# Autodesk Inventor assembly: Montagem1
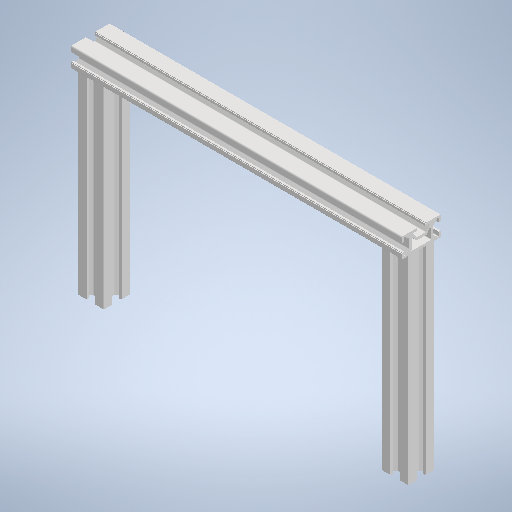
[picture p0: Inventor's stored thumbnail of the model, 512x512]
Saved by Autodesk Inventor 2025.2 (Build 292293000, 293)
## iProperties
Created: 2025-04-08
Part Number: Montagem1
Document SubType Name: Assembly
Designer: kenay
Author: kenay
## Documents named in this file (3)
- C:\Users\kenay\Downloads\Peças\Montagem1.iam
- C:\Users\kenay\Downloads\Peças\Peça3.ipt
- C:\Users\kenay\Downloads\Peças\Peça2.ipt
## Components (3 placed, 2 different names)
1. Peça2:1 — Coincidente:1, Alinhado:4, Coincidente:2, Alinhado:5
2. Peça3:1 — Alinhado:1, Alinhado:2, Alinhado:3, Coincidente:1, Alinhado:4, Alinhado:6, Alinhado:7
3. Peça3:2 — Coincidente:2, Alinhado:5, Alinhado:6, Alinhado:7
## Relationships (9: Flush 7, Mate 2)
- Alinhado:1 [Flush]: Peça3:1
- Alinhado:2 [Flush]: Peça3:1
- Alinhado:3 [Flush]: Peça3:1
- Coincidente:1 [Mate]: Peça2:1 ↔ Peça3:1
- Alinhado:4 [Flush]: Peça2:1 ↔ Peça3:1
- Coincidente:2 [Mate]: Peça2:1 ↔ Peça3:2
- Alinhado:5 [Flush]: Peça2:1 ↔ Peça3:2
- Alinhado:6 [Flush]: Peça3:1 ↔ Peça3:2
- Alinhado:7 [Flush]: Peça3:1 ↔ Peça3:2
